# Autodesk Inventor assembly: moisture housing
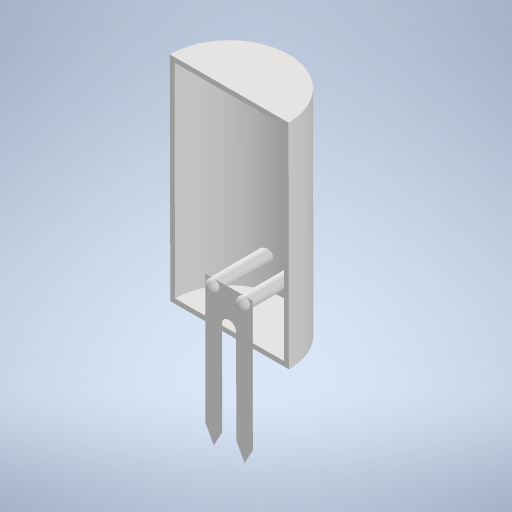
[picture p0: Inventor's stored thumbnail of the model, 512x512]
Saved by Autodesk Inventor 2023 (Build 270158000, 158)
## iProperties
Created: 2023-04-07
Part Number: moisture housing
Document SubType Name: Assembly
Designer: user
Author: user
## Documents named in this file (4)
- C:\Users\user\OneDrive\Desktop\projects\Robotics\smart farm\designs\moisture housing.iam
- C:\Users\user\OneDrive\Desktop\projects\Robotics\smart farm\designs\cover2.ipt
- C:\Users\user\OneDrive\Desktop\projects\Robotics\smart farm\designs\moisture sensor.ipt
- C:\Users\user\OneDrive\Desktop\projects\Robotics\smart farm\designs\screws.ipt
## Components (4 placed, 3 different names)
1. cover2:1 — Mate:1, Mate:2, Cylindrical:1, Rotation:1, Cylindrical:2
2. moisture sensor:1 — Mate:1, Mate:2
3. screws:1 — Cylindrical:1
4. screws:2 — Rotation:1, Cylindrical:2
## Relationships (5: Mate 2, CylindricalJoint 2, RelateRotation 1)
- Mate:1: cover2:1 ↔ moisture sensor:1
- Mate:2: cover2:1 ↔ moisture sensor:1
- Cylindrical:1: cover2:1 ↔ screws:1
- Rotation:1 [RelateRotation] (1 ul): cover2:1 ↔ screws:2
- Cylindrical:2: cover2:1 ↔ screws:2
